# Autodesk Inventor assembly: ENDER 3 ASSEMBLY
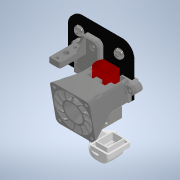
[picture p0: Inventor's stored thumbnail of the model, 180x180]
Saved by Autodesk Inventor 2022 (Build 260153070, 153G)
## iProperties
Created: 2022-01-01
Part Number: ENDER 3 ASSEMBLY
Document SubType Name: Assembly
Designer: a laptop
Author: a laptop
## Documents named in this file (12)
- C:\Users\a laptop\Desktop\Another3dPrinterShroud\MODELS\ENDER 3 ASSEMBLY.iam
- C:\Users\a laptop\Desktop\Another3dPrinterShroud\REF_MODEL\ENDER 3 E_PLATE.ipt
- C:\Users\a laptop\Desktop\Another3dPrinterShroud\REF_MODEL\ENDER 3 HEATBLOCK.ipt
- C:\Users\a laptop\Desktop\Another3dPrinterShroud\REF_MODEL\ENDER 3 HEATBREAK.ipt
- C:\Users\a laptop\Desktop\Another3dPrinterShroud\REF_MODEL\ENDER 3 RAD.ipt
- C:\Users\a laptop\Desktop\Another3dPrinterShroud\REF_MODEL\ENDER 3 NOZZLE.ipt
- C:\Users\a laptop\Desktop\Another3dPrinterShroud\REF_MODEL\ENDER 3 E_PLATE_SCREW.ipt
- C:\Users\a laptop\Desktop\Another3dPrinterShroud\MODELS\BACKPLATE.ipt
- C:\Users\a laptop\Desktop\Another3dPrinterShroud\MODELS\FRONTPLATE.ipt
- C:\Users\a laptop\Desktop\Another3dPrinterShroud\REF_MODEL\4020 AXIAL FAN.ipt
- C:\Users\a laptop\Desktop\Another3dPrinterShroud\REF_MODEL\5015 RADIAL FAN.ipt
- C:\Users\a laptop\Desktop\Another3dPrinterShroud\MODELS\DUCTV2.ipt
## Components (12 placed, 11 different names)
1. ENDER 3 E_PLATE:1 — Mate:1, Mate:2, Mate:3, Mate:11, Mate:12, Mate:14, Mate:15, Mate:16, Mate:17
2. ENDER 3 HEATBLOCK:1 — Mate:6, Mate:7, Mate:8, Flush:1, Flush:2
3. ENDER 3 HEATBREAK:1 — Mate:4, Mate:5, Mate:6, Mate:9, Mate:10
4. ENDER 3 RAD:1 — Mate:1, Mate:2, Mate:3, Mate:4, Mate:5, Mate:7, Mate:8, Angle:1
5. ENDER 3 NOZZLE:1 — Mate:9, Mate:10, Angle:1, Flush:1
6. ENDER 3 E_PLATE_SCREW:1 — Mate:11
7. ENDER 3 E_PLATE_SCREW:2 — Mate:12
8. BACKPLATE:1 — Mate:14, Mate:15
9. FRONTPLATE:1 — Flush:2, Mate:16, Mate:17, Mate:21, Mate:22, Mate:26, Mate:27, Mate:28, Mate:29
10. 4020 AXIAL FAN:1 — Mate:27, Mate:28, Mate:29
11. 5015 RADIAL FAN:2 — Mate:23, Mate:24, Mate:25
12. DUCTV2:1 — Mate:21, Mate:22, Mate:23, Mate:24, Mate:25, Mate:26
## Relationships (28: Mate 25, Flush 2, Angle 1)
- Mate:1: ENDER 3 E_PLATE:1 ↔ ENDER 3 RAD:1
- Mate:2: ENDER 3 E_PLATE:1 ↔ ENDER 3 RAD:1
- Mate:3: ENDER 3 E_PLATE:1 ↔ ENDER 3 RAD:1
- Mate:4: ENDER 3 HEATBREAK:1 ↔ ENDER 3 RAD:1
- Mate:5: ENDER 3 HEATBREAK:1 ↔ ENDER 3 RAD:1
- Mate:6: ENDER 3 HEATBLOCK:1 ↔ ENDER 3 HEATBREAK:1
- Mate:7: ENDER 3 HEATBLOCK:1 ↔ ENDER 3 RAD:1
- Mate:8: ENDER 3 HEATBLOCK:1 ↔ ENDER 3 RAD:1
- Mate:9: ENDER 3 HEATBREAK:1 ↔ ENDER 3 NOZZLE:1
- Mate:10: ENDER 3 HEATBREAK:1 ↔ ENDER 3 NOZZLE:1
- Angle:1 (0 deg): ENDER 3 RAD:1 ↔ ENDER 3 NOZZLE:1
- Flush:1: ENDER 3 HEATBLOCK:1 ↔ ENDER 3 NOZZLE:1
- Mate:11: ENDER 3 E_PLATE:1 ↔ ENDER 3 E_PLATE_SCREW:1
- Mate:12: ENDER 3 E_PLATE:1 ↔ ENDER 3 E_PLATE_SCREW:2
- Flush:2: ENDER 3 HEATBLOCK:1 ↔ FRONTPLATE:1
- Mate:14: ENDER 3 E_PLATE:1 ↔ BACKPLATE:1
- Mate:15: ENDER 3 E_PLATE:1 ↔ BACKPLATE:1
- Mate:16: ENDER 3 E_PLATE:1 ↔ FRONTPLATE:1
- Mate:17: ENDER 3 E_PLATE:1 ↔ FRONTPLATE:1
- Mate:21: FRONTPLATE:1 ↔ DUCTV2:1
- Mate:22: FRONTPLATE:1 ↔ DUCTV2:1
- Mate:23: 5015 RADIAL FAN:2 ↔ DUCTV2:1
- Mate:24: 5015 RADIAL FAN:2 ↔ DUCTV2:1
- Mate:25: 5015 RADIAL FAN:2 ↔ DUCTV2:1
- Mate:26: FRONTPLATE:1 ↔ DUCTV2:1
- Mate:27: FRONTPLATE:1 ↔ 4020 AXIAL FAN:1
- Mate:28: FRONTPLATE:1 ↔ 4020 AXIAL FAN:1
- Mate:29: FRONTPLATE:1 ↔ 4020 AXIAL FAN:1
